# Autodesk Inventor assembly: Moduł_hamujący
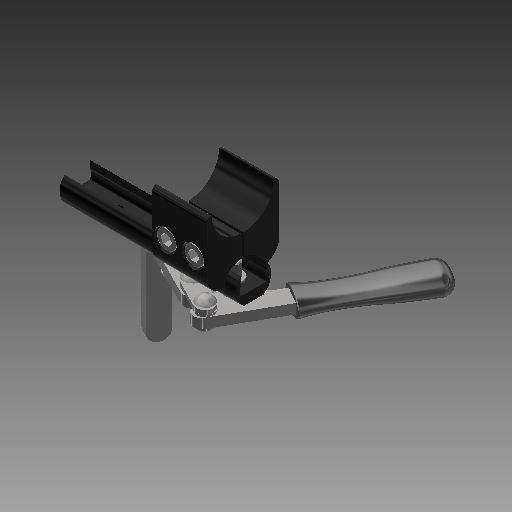
[picture p0: Inventor's stored thumbnail of the model, 512x512]
Saved by Autodesk Inventor 2017 (Build 210142000, 142)
## iProperties
Created: 2015-12-05
Part Number: Moduł_hamujący
Document SubType Name: Assembly
Designer: graaapsik
Author: graaapsik
## Documents named in this file (13)
- D:\Documents\Centro Universitário da FEI\Wheelchair\CADEIRA DE RODAS - DESENHO\GITHUB\Hamulec.iam
- D:\Documents\Centro Universitário da FEI\Wheelchair\CADEIRA DE RODAS - DESENHO\GITHUB\Pręt_cierny.ipt
- D:\Documents\Centro Universitário da FEI\Wheelchair\CADEIRA DE RODAS - DESENHO\GITHUB\ISO 7092 - ST 5 - 140 HV.ipt
- D:\Documents\Centro Universitário da FEI\Wheelchair\CADEIRA DE RODAS - DESENHO\GITHUB\ISO_R 1051 - 5 x 22 x 10.ipt
- D:\Documents\Centro Universitário da FEI\Wheelchair\CADEIRA DE RODAS - DESENHO\GITHUB\Łącznik.ipt
- D:\Documents\Centro Universitário da FEI\Wheelchair\CADEIRA DE RODAS - DESENHO\GITHUB\Dźwignia.ipt
- D:\Documents\Centro Universitário da FEI\Wheelchair\CADEIRA DE RODAS - DESENHO\GITHUB\Pasek_regulacji.ipt
- D:\Documents\Centro Universitário da FEI\Wheelchair\CADEIRA DE RODAS - DESENHO\GITHUB\Zawias.ipt
- D:\Documents\Centro Universitário da FEI\Wheelchair\CADEIRA DE RODAS - DESENHO\GITHUB\ISO 4762 - M6 x 30ISO.ipt
- D:\Documents\Centro Universitário da FEI\Wheelchair\CADEIRA DE RODAS - DESENHO\GITHUB\ISO 7092 - ST 6 - 140 HV.ipt
- D:\Documents\Centro Universitário da FEI\Wheelchair\CADEIRA DE RODAS - DESENHO\GITHUB\ISO 7380 - M6 x 20.ipt
- D:\Documents\Centro Universitário da FEI\Wheelchair\CADEIRA DE RODAS - DESENHO\GITHUB\ISO 4035 - M6ISO.ipt
- D:\Documents\Centro Universitário da FEI\Wheelchair\CADEIRA DE RODAS - DESENHO\GITHUB\Osłona_dźwigni.ipt
## Components (29 placed, 12 different names)
1. Zawias:1 — Zestawiający:40, Zestawiający:41, Zestawiający:42, Zestawiający:51, Wstaw:5, Wstaw:6
2. Zawias:2 — Zestawiający:40, Zestawiający:41, Zestawiający:42, Kąt:1, Równoległy:1, Wstaw:1, Wstaw:2
3. Pasek_regulacji:1 — Zestawiający:51, Kąt:1, Równoległy:1, Wstaw:17, Wstaw:18, Wstaw:19, Wstaw:20
4. Pręt_cierny:1 — Zestawiający:74, Zestawiający:75, Zestawiający:79, Zestawiający:80, Zestawiający:82
5. ISO_R 1051 - 5 x 22 x 10:1 — Zestawiający:11, Wstaw:10, Zestawiający:75, Zestawiający:76
6. Łącznik:1 — Zestawiający:11, Zestawiający:24, Zestawiający:81
7. Dźwignia:1 — Zestawiający:18, Zestawiający:28, Zestawiający:63, Zestawiający:64, Zestawiający:65, Wstaw:11, Wstaw:14, Zestawiający:73, Zestawiający:78
8. ISO_R 1051 - 5 x 22 x 10:2 — Zestawiający:18, Zestawiający:24, Zestawiający:28, Wstaw:9
9. Osłona_dźwigni:1 — Zestawiający:63, Zestawiający:64, Zestawiający:65
10. ISO 4035 M6:3 — Wstaw:8
11. ISO 7092 ST 6 - 140 HV:5 — Wstaw:1, Wstaw:3
12. ISO 4762 M6 x 30:3 — Wstaw:3
13. ISO 4762 M6 x 30:4 — Wstaw:4
14. ISO 7092 ST 6 - 140 HV:6 — Wstaw:2, Wstaw:4
15. ISO 7092 ST 6 - 140 HV:7 — Wstaw:6, Wstaw:8
16. ISO 7092 ST 6 - 140 HV:8 — Wstaw:5, Wstaw:7
17. ISO 4035 M6:4 — Wstaw:7
18. ISO 7380 M6 x 20:3 — Wstaw:16, Zestawiający:67
19. ISO 7380 M6 x 20:4 — Wstaw:15, Zestawiający:66, Zestawiający:74
20. ISO 7092 ST 5 - 140 HV:11 — Wstaw:10, Zestawiający:80
21. ISO 7092 ST 5 - 140 HV:12 — Wstaw:9, Zestawiający:73
22. ISO 7092 ST 5 - 140 HV:13 — Wstaw:11, Zestawiający:81
23. ISO 7092 ST 5 - 140 HV:14 — Zestawiający:76, Zestawiający:82
24. ISO 7092 ST 5 - 140 HV:15 — Wstaw:14, Wstaw:16
25. ISO 7092 ST 5 - 140 HV:16 — Wstaw:15
26. ISO 7092 ST 5 - 140 HV:17 — Wstaw:17, Zestawiający:67, Zestawiający:78
27. ISO 7092 ST 5 - 140 HV:18 — Wstaw:19
28. ISO 7092 ST 5 - 140 HV:19 — Wstaw:20, Zestawiający:66, Zestawiający:79
29. ISO 7092 ST 5 - 140 HV:20 — Wstaw:18
## Relationships (42: Mate 22, Insert 18, Angle 1, Flush 1)
- Zestawiający:11 [Mate]: ISO_R 1051 - 5 x 22 x 10:1 ↔ Łącznik:1
- Zestawiający:18 [Mate]: Dźwignia:1 ↔ ISO_R 1051 - 5 x 22 x 10:2
- Zestawiający:24 [Mate]: Łącznik:1 ↔ ISO_R 1051 - 5 x 22 x 10:2
- Zestawiający:28 [Mate]: Dźwignia:1 ↔ ISO_R 1051 - 5 x 22 x 10:2
- Zestawiający:40 [Mate] (1 mm): Zawias:1 ↔ Zawias:2
- Zestawiający:41 [Mate]: Zawias:1 ↔ Zawias:2
- Zestawiający:42 [Mate]: Zawias:1 ↔ Zawias:2
- Zestawiający:51 [Mate]: Zawias:1 ↔ Pasek_regulacji:1
- Kąt:1 [Angle] (90 deg): Zawias:2 ↔ Pasek_regulacji:1
- Równoległy:1 [Flush] (-5 mm): Zawias:2 ↔ Pasek_regulacji:1
- Zestawiający:63 [Mate]: Dźwignia:1 ↔ Osłona_dźwigni:1
- Zestawiający:64 [Mate]: Dźwignia:1 ↔ Osłona_dźwigni:1
- Zestawiający:65 [Mate]: Dźwignia:1 ↔ Osłona_dźwigni:1
- Wstaw:1 [Insert]: Zawias:2 ↔ ISO 7092 ST 6 - 140 HV:5
- Wstaw:2 [Insert]: Zawias:2 ↔ ISO 7092 ST 6 - 140 HV:6
- Wstaw:3 [Insert]: ISO 7092 ST 6 - 140 HV:5 ↔ ISO 4762 M6 x 30:3
- Wstaw:4 [Insert]: ISO 4762 M6 x 30:4 ↔ ISO 7092 ST 6 - 140 HV:6
- Wstaw:5 [Insert]: Zawias:1 ↔ ISO 7092 ST 6 - 140 HV:8
- Wstaw:6 [Insert]: Zawias:1 ↔ ISO 7092 ST 6 - 140 HV:7
- Wstaw:7 [Insert]: ISO 7092 ST 6 - 140 HV:8 ↔ ISO 4035 M6:4
- Wstaw:8 [Insert]: ISO 4035 M6:3 ↔ ISO 7092 ST 6 - 140 HV:7
- Wstaw:9 [Insert]: ISO_R 1051 - 5 x 22 x 10:2 ↔ ISO 7092 ST 5 - 140 HV:12
- Wstaw:10 [Insert]: ISO_R 1051 - 5 x 22 x 10:1 ↔ ISO 7092 ST 5 - 140 HV:11
- Wstaw:11 [Insert]: Dźwignia:1 ↔ ISO 7092 ST 5 - 140 HV:13
- Wstaw:14 [Insert]: Dźwignia:1 ↔ ISO 7092 ST 5 - 140 HV:15
- Wstaw:15 [Insert]: ISO 7380 M6 x 20:4 ↔ ISO 7092 ST 5 - 140 HV:16
- Wstaw:16 [Insert]: ISO 7380 M6 x 20:3 ↔ ISO 7092 ST 5 - 140 HV:15
- Wstaw:17 [Insert]: Pasek_regulacji:1 ↔ ISO 7092 ST 5 - 140 HV:17
- Wstaw:18 [Insert]: Pasek_regulacji:1 ↔ ISO 7092 ST 5 - 140 HV:20
- Wstaw:19 [Insert]: Pasek_regulacji:1 ↔ ISO 7092 ST 5 - 140 HV:18
- Wstaw:20 [Insert]: Pasek_regulacji:1 ↔ ISO 7092 ST 5 - 140 HV:19
- Zestawiający:66 [Mate]: ISO 7380 M6 x 20:4 ↔ ISO 7092 ST 5 - 140 HV:19
- Zestawiający:67 [Mate]: ISO 7380 M6 x 20:3 ↔ ISO 7092 ST 5 - 140 HV:17
- Zestawiający:73 [Mate]: Dźwignia:1 ↔ ISO 7092 ST 5 - 140 HV:12
- Zestawiający:74 [Mate]: Pręt_cierny:1 ↔ ISO 7380 M6 x 20:4
- Zestawiający:75 [Mate]: Pręt_cierny:1 ↔ ISO_R 1051 - 5 x 22 x 10:1
- Zestawiający:76 [Mate]: ISO_R 1051 - 5 x 22 x 10:1 ↔ ISO 7092 ST 5 - 140 HV:14
- Zestawiający:78 [Mate]: Dźwignia:1 ↔ ISO 7092 ST 5 - 140 HV:17
- Zestawiający:79 [Mate]: Pręt_cierny:1 ↔ ISO 7092 ST 5 - 140 HV:19
- Zestawiający:80 [Mate]: Pręt_cierny:1 ↔ ISO 7092 ST 5 - 140 HV:11
- Zestawiający:81 [Mate]: Łącznik:1 ↔ ISO 7092 ST 5 - 140 HV:13
- Zestawiający:82 [Mate]: Pręt_cierny:1 ↔ ISO 7092 ST 5 - 140 HV:14
